# Autodesk Inventor assembly: robot arm box
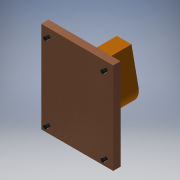
[picture p0: Inventor's stored thumbnail of the model, 180x180]
Saved by Autodesk Inventor 2018 (Build 220112000, 112)
## iProperties
Created: 2017-10-09
Part Number: robot arm box
Document SubType Name: Assembly
Designer: HP
Author: HP
## Documents named in this file (2)
- C:\!_Dani\!_cloud\ownCloud\rover\Robot arm box\robot arm box.iam
- C:\!_Dani\!_cloud\ownCloud\rover\Robot arm box\basic plate.ipt
## Components (1 placed, 1 different names)
1. basic plate:1 — Flush:2, Mate:1, Mate:2
## Relationships (3: Mate 2, Flush 1)
- Flush:2: basic plate:1
- Mate:1: basic plate:1
- Mate:2: basic plate:1
